# Autodesk Inventor assembly: Colossus_7kW
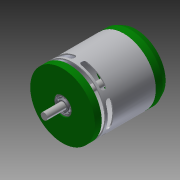
[picture p0: Inventor's stored thumbnail of the model, 180x180]
Saved by Autodesk Inventor 2014 (Build 180170000, 170)
## iProperties
Created: 2014-11-23
Part Number: Colossus_7kW
Document SubType Name: Assembly
Designer: Yann
Author: Yann
## Documents named in this file (6)
- C:\Users\Yann\Documents\GitHub\BIKAIR_CAD\Source\Motor\Motor.iam
- C:\Users\Yann\Documents\GitHub\BIKAIR_CAD\Source\Motor\Motor_Stator.ipt
- C:\Users\Yann\Documents\GitHub\BIKAIR_CAD\Source\Motor\Motor_Rotor.ipt
- C:\Users\Yann\Documents\GitHub\BIKAIR_CAD\Source\Motor\Motor_Rotor_body.ipt
- C:\Users\Yann\Documents\GitHub\BIKAIR_CAD\Source\Motor\Motor_Shaft.ipt
- C:\Users\Yann\Documents\GitHub\BIKAIR_CAD\Source\Motor\ANSI_AFBMA 16.1 - 12 x 32 x 16.ipt
## Components (6 placed, 5 different names)
1. Motor_Stator:1 — Affleurement:1, Affleurement:2, Affleurement:3, Rotation:1
2. Motor_Rotor:1 — Affleurement:4, Affleurement:5, Affleurement:6, Placage:1, Placage:2, Rotation:2
3. Motor_Rotor_body:1 — Affleurement:7, Affleurement:8, Placage:1
4. Motor_Shaft:1 — Affleurement:9, Affleurement:10, Placage:2
5. ANSI/AFBMA 16.1 - Roulements à billes aéro: deux rangées, fixe, diamètre de série 2 12 x 32 x 16:1 — Rotation:2
6. ANSI/AFBMA 16.1 - Roulements à billes aéro: deux rangées, fixe, diamètre de série 2 12 x 32 x 16:2 — Rotation:1
## Relationships (14: Flush 10, Mate 2, RevoluteJoint 2)
- Affleurement:1 [Flush]: Motor_Stator:1
- Affleurement:2 [Flush]: Motor_Stator:1
- Affleurement:3 [Flush]: Motor_Stator:1
- Affleurement:4 [Flush]: Motor_Rotor:1
- Affleurement:5 [Flush]: Motor_Rotor:1
- Affleurement:6 [Flush] (130 mm): Motor_Rotor:1
- Affleurement:7 [Flush]: Motor_Rotor_body:1
- Affleurement:8 [Flush]: Motor_Rotor_body:1
- Placage:1 [Mate]: Motor_Rotor:1 ↔ Motor_Rotor_body:1
- Affleurement:9 [Flush]: Motor_Shaft:1
- Affleurement:10 [Flush]: Motor_Shaft:1
- Placage:2 [Mate]: Motor_Rotor:1 ↔ Motor_Shaft:1
- Rotation:1 [RevoluteJoint]: Motor_Stator:1 ↔ ANSI/AFBMA 16.1 - Roulements à billes aéro: deux rangées, fixe, diamètre de série 2 12 x 32 x 16:2
- Rotation:2 [RevoluteJoint]: Motor_Rotor:1 ↔ ANSI/AFBMA 16.1 - Roulements à billes aéro: deux rangées, fixe, diamètre de série 2 12 x 32 x 16:1
